# Autodesk Inventor assembly: VersaPlanetary Dual Input BAG
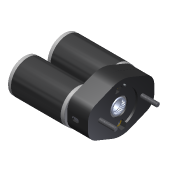
[picture p0: Inventor's stored thumbnail of the model, 180x180]
Saved by Autodesk Inventor 2013 (Build 170138000, 138)
## iProperties
Created: 2013-12-15
Part Number: VersaPlanetary Dual Input BAG
Document SubType Name: Assembly
Designer: Nemo
Author: Nemo
## Documents named in this file (13)
- \\lmss\students\Robotics\CAD Files\COTS Parts\VersaPlanetary\VersaPlanetary Dual Input BAG.iam
- \\lmss\students\Robotics\CAD Files\COTS Parts\VersaPlanetary\Components\VersaPlanetary Dual Input output side casing.ipt
- \\lmss\students\Robotics\CAD Files\COTS Parts\Bearings - VexPro\Radial Bearing - 17mm x 26mm x 5mm.ipt
- \\lmss\students\Robotics\CAD Files\COTS Parts\VersaPlanetary\Components\VersaPlanetary Dual Input motor side casing.ipt
- \\lmss\students\Robotics\CAD Files\COTS Parts\VersaPlanetary\Components\VersaPlanetary Dual Input output gear.ipt
- \\lmss\students\Robotics\CAD Files\COTS Parts\VersaPlanetary\Components\VersaPlanetary Dual Input input gear.ipt
- \\lmss\students\Robotics\CAD Files\COTS Parts\Fasteners\10-32 SHCS x875.ipt
- \\lmss\students\Robotics\CAD Files\COTS Parts\Fasteners\8-32 SHCS x750.ipt
- \\lmss\students\Robotics\CAD Files\COTS Parts\Fasteners\8-32 locknut.ipt
- \\lmss\students\Robotics\CAD Files\COTS Parts\VersaPlanetary\Components\VersaPlanetary BAG shaft piece.ipt
- \\lmss\students\Robotics\CAD Files\COTS Parts\Motors\BAG Motor.ipt
- \\lmss\students\Robotics\CAD Files\COTS Parts\Fasteners\M4 SHCS x10.ipt
- \\lmss\students\Robotics\CAD Files\COTS Parts\VersaPlanetary\Components\VersaPlanetary pin.ipt
## Components (22 placed, 12 different names)
1. VersaPlanetary Dual Input output side casing:1 — Insert:1, Mate:1, Mate:2, Insert:4, Insert:5, Mate:5, Insert:8, Insert:9, Insert:18, Mate:10, Mate:11, Flush:1
2. Radial Bearing - 17mm x 26mm x 5mm:1 — Insert:2
3. Radial Bearing - 17mm x 26mm x 5mm:2 — Insert:1, Insert:3
4. VersaPlanetary Dual Input motor side casing:1 — Mate:1, Insert:2, Mate:2, Mate:3, Mate:4, Mate:5, Mate:6, Mate:7, Insert:6, Insert:7, Insert:12, Insert:13, Insert:14, Insert:15, Insert:16, Insert:17
5. VersaPlanetary Dual Input output gear:1 — Insert:3
6. VersaPlanetary Dual Input input gear:1 — Mate:4, Mate:6, Insert:11
7. VersaPlanetary Dual Input input gear:2 — Mate:3, Mate:7, Insert:10
8. 10-32 SHCS x875:1 — Insert:5
9. 10-32 SHCS x875:2 — Insert:4
10. 8-32 SHCS x750:1 — Insert:6
11. 8-32 SHCS x750:2 — Insert:7
12. 8-32 locknut:1 — Insert:9
13. 8-32 locknut:2 — Insert:8
14. VersaPlanetary BAG shaft piece:1 — Insert:10
15. VersaPlanetary BAG shaft piece:2 — Insert:11
16. BAG Motor:1 — Insert:17, Mate:9
17. BAG Motor:2 — Insert:16, Mate:8
18. M4 SHCS x10:1 — Insert:13
19. M4 SHCS x10:2 — Insert:14, Mate:9
20. M4 SHCS x10:3 — Insert:15, Mate:8
21. M4 SHCS x10:4 — Insert:12
22. VersaPlanetary pin:1 — Insert:18
## Relationships (30: Insert 18, Mate 11, Flush 1)
- Insert:1: VersaPlanetary Dual Input output side casing:1 ↔ Radial Bearing - 17mm x 26mm x 5mm:2
- Mate:1: VersaPlanetary Dual Input output side casing:1 ↔ VersaPlanetary Dual Input motor side casing:1
- Insert:2: Radial Bearing - 17mm x 26mm x 5mm:1 ↔ VersaPlanetary Dual Input motor side casing:1
- Insert:3: Radial Bearing - 17mm x 26mm x 5mm:2 ↔ VersaPlanetary Dual Input output gear:1
- Mate:2: VersaPlanetary Dual Input output side casing:1 ↔ VersaPlanetary Dual Input motor side casing:1
- Mate:3: VersaPlanetary Dual Input motor side casing:1 ↔ VersaPlanetary Dual Input input gear:2
- Mate:4: VersaPlanetary Dual Input motor side casing:1 ↔ VersaPlanetary Dual Input input gear:1
- Insert:4: VersaPlanetary Dual Input output side casing:1 ↔ 10-32 SHCS x875:2
- Insert:5: VersaPlanetary Dual Input output side casing:1 ↔ 10-32 SHCS x875:1
- Mate:5: VersaPlanetary Dual Input output side casing:1 ↔ VersaPlanetary Dual Input motor side casing:1
- Mate:6: VersaPlanetary Dual Input motor side casing:1 ↔ VersaPlanetary Dual Input input gear:1
- Mate:7: VersaPlanetary Dual Input motor side casing:1 ↔ VersaPlanetary Dual Input input gear:2
- Insert:6: VersaPlanetary Dual Input motor side casing:1 ↔ 8-32 SHCS x750:1
- Insert:7: VersaPlanetary Dual Input motor side casing:1 ↔ 8-32 SHCS x750:2
- Insert:8: VersaPlanetary Dual Input output side casing:1 ↔ 8-32 locknut:2
- Insert:9: VersaPlanetary Dual Input output side casing:1 ↔ 8-32 locknut:1
- Insert:10: VersaPlanetary Dual Input input gear:2 ↔ VersaPlanetary BAG shaft piece:1
- Insert:11: VersaPlanetary Dual Input input gear:1 ↔ VersaPlanetary BAG shaft piece:2
- Insert:12: VersaPlanetary Dual Input motor side casing:1 ↔ M4 SHCS x10:4
- Insert:13: VersaPlanetary Dual Input motor side casing:1 ↔ M4 SHCS x10:1
- Insert:14: VersaPlanetary Dual Input motor side casing:1 ↔ M4 SHCS x10:2
- Insert:15: VersaPlanetary Dual Input motor side casing:1 ↔ M4 SHCS x10:3
- Insert:16: VersaPlanetary Dual Input motor side casing:1 ↔ BAG Motor:2
- Mate:8: BAG Motor:2 ↔ M4 SHCS x10:3
- Insert:17: VersaPlanetary Dual Input motor side casing:1 ↔ BAG Motor:1
- Mate:9: BAG Motor:1 ↔ M4 SHCS x10:2
- Insert:18: VersaPlanetary Dual Input output side casing:1 ↔ VersaPlanetary pin:1
- Mate:10: VersaPlanetary Dual Input output side casing:1
- Mate:11: VersaPlanetary Dual Input output side casing:1
- Flush:1: VersaPlanetary Dual Input output side casing:1
